# Autodesk Inventor assembly: A2017_T4_12
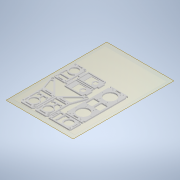
[picture p0: Inventor's stored thumbnail of the model, 180x180]
Saved by Autodesk Inventor 2020 (Build 240168000, 168)
## iProperties
Created: 2021-08-27
Part Number: A2017_T4_12
Document SubType Name: Assembly
Designer: Masato
Author: Masato
## Documents named in this file (7)
- C:\Inventor\SUSTAINA-OP\Cam\A2017_T4_12.iam
- C:\Inventor\SUSTAINA-OP\Cam\DisposableBoard.ipt
- C:\Inventor\SUSTAINA-OP\UpperBody\Trunk\Trunk_neck_frame.ipt
- C:\Inventor\SUSTAINA-OP\UpperBody\Trunk\Trunk_shoulder_frame.ipt
- C:\Inventor\SUSTAINA-OP\UpperBody\Trunk\Trunk_shoulder_frame_MIR.ipt
- C:\Inventor\SUSTAINA-OP\UpperBody\Trunk\Trunk_waisit_frame.ipt
- C:\Inventor\SUSTAINA-OP\UpperBody\Trunk\Trunk_servo_bottom_frame.ipt
## Components (8 placed, 6 different names)
1. DisposableBoard:1 — メイト:2, メイト:1, フラッシュ:1, フラッシュ:2, メイト:10, メイト:11, フラッシュ:3, 正接:1, メイト:12, メイト:15, メイト:17, フラッシュ:6, メイト:18
2. Trunk_neck_frame:2 — メイト:10, メイト:14, フラッシュ:5, メイト:16
3. Trunk_shoulder_frame:1 — メイト:11, フラッシュ:3, 正接:1, フラッシュ:4, メイト:13, フラッシュ:5, 正接:3
4. Trunk_shoulder_frame_MIR:1 — メイト:12, フラッシュ:4, メイト:13, メイト:14, 正接:2, メイト:20
5. Trunk_waisit_frame:1 — メイト:15, メイト:16, 正接:2
6. Trunk_neck_frame:3 — メイト:17, フラッシュ:6, 正接:3, メイト:19
7. Trunk_servo_bottom_frame:1 — メイト:18, メイト:19, メイト:20
8. Trunk_servo_bottom_frame:2
## Component patterns: (2 elements, first: Trunk_servo_bottom_frame:1)
## Relationships (22: Mate 13, Flush 6, Tangent 3)
- メイト:2 [Mate]: DisposableBoard:1
- メイト:1 [Mate]: DisposableBoard:1
- フラッシュ:1 [Flush]: DisposableBoard:1
- フラッシュ:2 [Flush]: DisposableBoard:1
- メイト:10 [Mate]: DisposableBoard:1 ↔ Trunk_neck_frame:2
- メイト:11 [Mate]: DisposableBoard:1 ↔ Trunk_shoulder_frame:1
- フラッシュ:3 [Flush] (2 mm): DisposableBoard:1 ↔ Trunk_shoulder_frame:1
- 正接:1 [Tangent] (2 mm): DisposableBoard:1 ↔ Trunk_shoulder_frame:1
- メイト:12 [Mate]: DisposableBoard:1 ↔ Trunk_shoulder_frame_MIR:1
- フラッシュ:4 [Flush]: Trunk_shoulder_frame:1 ↔ Trunk_shoulder_frame_MIR:1
- メイト:13 [Mate] (2.5 mm): Trunk_shoulder_frame:1 ↔ Trunk_shoulder_frame_MIR:1
- メイト:14 [Mate] (2.5 mm): Trunk_neck_frame:2 ↔ Trunk_shoulder_frame_MIR:1
- フラッシュ:5 [Flush]: Trunk_neck_frame:2 ↔ Trunk_shoulder_frame:1
- メイト:15 [Mate]: DisposableBoard:1 ↔ Trunk_waisit_frame:1
- メイト:16 [Mate] (2.5 mm): Trunk_neck_frame:2 ↔ Trunk_waisit_frame:1
- 正接:2 [Tangent] (2.5 mm): Trunk_shoulder_frame_MIR:1 ↔ Trunk_waisit_frame:1
- メイト:17 [Mate]: DisposableBoard:1 ↔ Trunk_neck_frame:3
- フラッシュ:6 [Flush] (2 mm): DisposableBoard:1 ↔ Trunk_neck_frame:3
- 正接:3 [Tangent] (2.5 mm): Trunk_shoulder_frame:1 ↔ Trunk_neck_frame:3
- メイト:18 [Mate]: DisposableBoard:1 ↔ Trunk_servo_bottom_frame:1
- メイト:19 [Mate] (2.5 mm): Trunk_neck_frame:3 ↔ Trunk_servo_bottom_frame:1
- メイト:20 [Mate] (2.5 mm): Trunk_shoulder_frame_MIR:1 ↔ Trunk_servo_bottom_frame:1
